# Autodesk Inventor assembly: main_assembly
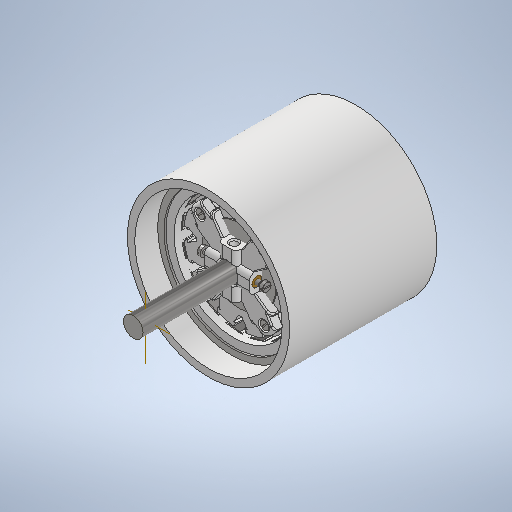
[picture p0: Inventor's stored thumbnail of the model, 512x512]
Saved by Autodesk Inventor 2025 (Build 290162000, 162)
## iProperties
Created: 2026-08-03
Part Number: main_assembly
Document SubType Name: Assembly
Designer: zzapa
Author: zzapa
## Documents named in this file (13)
- C:\Users\zzapa\Desktop\Projekty\elektronika\engine-project\model\assemblies\main_assembly.iam
- C:\Users\zzapa\Desktop\Projekty\elektronika\engine-project\model\parts\stator_metal.ipt
- C:\Users\zzapa\Desktop\Projekty\elektronika\engine-project\model\assemblies\magnet_ring_assembly.iam
- C:\Users\zzapa\Desktop\Projekty\elektronika\engine-project\model\parts\casing_cylindrical.ipt
- C:\Users\zzapa\Desktop\Projekty\elektronika\engine-project\model\parts\rotor_plastic.ipt
- C:\Users\zzapa\Desktop\Projekty\elektronika\engine-project\model\assemblies\rotor_core.iam
- C:\Users\zzapa\Desktop\Projekty\elektronika\engine-project\model\parts\shaft.ipt
- C:\Users\zzapa\Documents\Inventor\Content Center Files\R2025\pl-PL\GB 809-88 A\Nut GB 809 A M2,5 x 6.ipt
- C:\Users\zzapa\Documents\Inventor\Content Center Files\R2025\pl-PL\CNS 4355\CNS 4355 - M 2 x 6.ipt
- C:\Users\zzapa\Desktop\Projekty\elektronika\engine-project\model\parts\shaft_lock_1.ipt
- C:\Users\zzapa\Documents\Inventor\Content Center Files\R2025\pl-PL\GB 809-88 A\Nut GB 809 A M2 x 3.ipt
- C:\Users\zzapa\Documents\Inventor\Content Center Files\R2025\pl-PL\CNS 4355\CNS 4355 - M 2 x 8.ipt
- C:\Users\zzapa\Desktop\Projekty\elektronika\engine-project\model\parts\shaft_lock_2.ipt
## Components (32 placed, 12 different names)
1. stator_metal:1 — Zestawiające:1, Kątowe:1
2. magnet_ring_assembly:1 [sub-assembly] — Zestawiające:2
3. casing_cylindrical:1 — Zestawiające:3, Kątowe:2
4. rotor_plastic:1 — Zestawiające:4, Zestawiające:7, Zestawiające:8, Zestawiające:9, Zestawiające:10, Równoległe:1, Równoległe:2, Równoległe:3, Równoległe:4, Zestawiające:31, Zestawiające:40, Zestawiające:41, Zestawiające:42, Zestawiające:43, Zestawiające:44, Równoległe:5, Równoległe:6, Równoległe:7, Równoległe:8, Kątowe:13, Zestawiające:52
5. rotor_core:1 [sub-assembly] — Zestawiające:5, Zestawiające:30
6. shaft:1 — Zestawiające:6, Zestawiające:28, Styczny:1, Styczny:2, Zestawiające:50
7. Nut GB/T 809-1988 Type A M2,5x6:1 — Kątowe:3, Zestawiające:7, Równoległe:3
8. Nut GB/T 809-1988 Type A M2,5x6:2 — Kątowe:4, Zestawiające:9, Równoległe:1
9. Nut GB/T 809-1988 Type A M2,5x6:3 — Kątowe:5, Zestawiające:8, Równoległe:2, Zestawiające:51
10. Nut GB/T 809-1988 Type A M2,5x6:4 — Kątowe:6, Zestawiające:10, Równoległe:4
11. shaft_lock_1:1 — Zestawiające:28, Zestawiające:30, Zestawiające:31, Zestawiające:32, Zestawiające:33, Zestawiające:34, Zestawiające:35, Zestawiające:36, Zestawiające:37, Zestawiające:38, Zestawiające:39, Zestawiające:40, Zestawiające:45, Zestawiające:46, Równoległe:9, Równoległe:10
12. CNS 4355 M 2 x 6:5 — Zestawiające:32, Zestawiające:36
13. CNS 4355 M 2 x 6:6 — Zestawiające:35, Zestawiające:39
14. CNS 4355 M 2 x 6:7 — Zestawiające:34, Zestawiające:38
15. CNS 4355 M 2 x 6:8 — Zestawiające:33, Zestawiające:37
16. Nut GB/T 809-1988 Type A M2,5x6:6 — Zestawiające:42, Równoległe:7
17. Nut GB/T 809-1988 Type A M2,5x6:7 — Zestawiające:44, Równoległe:6
18. Nut GB/T 809-1988 Type A M2,5x6:8 — Zestawiające:43, Równoległe:5
19. Nut GB/T 809-1988 Type A M2,5x6:9 — Zestawiające:41, Równoległe:8
20. Nut GB/T 809-1988 Type A M2x3:1 — Zestawiające:45, Równoległe:10, Zestawiające:47
21. Nut GB/T 809-1988 Type A M2x3:2 — Zestawiające:46, Równoległe:9, Zestawiające:48
22. CNS 4355 M 2 x 8:1 — Zestawiające:48, Równoległe:11
23. CNS 4355 M 2 x 8:2 — Zestawiające:47, Zestawiające:49
24. shaft_lock_2:1 — Zestawiające:50, Zestawiające:51, Zestawiające:52, Zestawiające:53, Zestawiające:54, Równoległe:12, Równoległe:13, Zestawiające:58, Zestawiające:59, Zestawiające:60, Zestawiające:61, Zestawiające:62, Zestawiające:63, Zestawiające:64, Zestawiające:65
25. Nut GB/T 809-1988 Type A M2x3:3 — Zestawiające:53, Równoległe:13, Zestawiające:57
26. Nut GB/T 809-1988 Type A M2x3:4 — Zestawiające:54, Równoległe:12, Zestawiające:56
27. CNS 4355 M 2 x 8:3 — Zestawiające:55, Zestawiające:57
28. CNS 4355 M 2 x 8:4 — Równoległe:14, Zestawiające:56
29. CNS 4355 M 2 x 6:9 — Zestawiające:60, Zestawiające:63
30. CNS 4355 M 2 x 6:10 — Zestawiające:61, Zestawiające:64
31. CNS 4355 M 2 x 6:11 — Zestawiające:59, Zestawiające:65
32. CNS 4355 M 2 x 6:12 — Zestawiające:58, Zestawiające:62
## Relationships (72: Mate 47, Flush 14, Angle 9, Tangent 2)
- Zestawiające:1 [Mate]: stator_metal:1
- Kątowe:1 [Angle] (0 deg): stator_metal:1
- Zestawiające:2 [Mate]: magnet_ring_assembly:1
- Zestawiające:3 [Mate]: casing_cylindrical:1
- Kątowe:2 [Angle] (0 deg): casing_cylindrical:1
- Zestawiające:4 [Mate]: rotor_plastic:1
- Zestawiające:5 [Mate]: rotor_core:1
- Zestawiające:6 [Mate]: shaft:1
- Kątowe:3 [Angle] (0 deg): Nut GB/T 809-1988 Type A M2,5x6:1
- Kątowe:4 [Angle] (0 deg): Nut GB/T 809-1988 Type A M2,5x6:2
- Kątowe:5 [Angle] (0 deg): Nut GB/T 809-1988 Type A M2,5x6:3
- Kątowe:6 [Angle] (0 deg): Nut GB/T 809-1988 Type A M2,5x6:4
- Zestawiające:7 [Mate]: rotor_plastic:1 ↔ Nut GB/T 809-1988 Type A M2,5x6:1
- Zestawiające:8 [Mate]: rotor_plastic:1 ↔ Nut GB/T 809-1988 Type A M2,5x6:3
- Zestawiające:9 [Mate]: rotor_plastic:1 ↔ Nut GB/T 809-1988 Type A M2,5x6:2
- Zestawiające:10 [Mate]: rotor_plastic:1 ↔ Nut GB/T 809-1988 Type A M2,5x6:4
- Równoległe:1 [Flush]: rotor_plastic:1 ↔ Nut GB/T 809-1988 Type A M2,5x6:2
- Równoległe:2 [Flush]: rotor_plastic:1 ↔ Nut GB/T 809-1988 Type A M2,5x6:3
- Równoległe:3 [Flush]: rotor_plastic:1 ↔ Nut GB/T 809-1988 Type A M2,5x6:1
- Równoległe:4 [Flush]: rotor_plastic:1 ↔ Nut GB/T 809-1988 Type A M2,5x6:4
- Zestawiające:28 [Mate]: shaft:1 ↔ shaft_lock_1:1
- Zestawiające:30 [Mate]: rotor_core:1 ↔ shaft_lock_1:1
- Zestawiające:31 [Mate]: rotor_plastic:1 ↔ shaft_lock_1:1
- Zestawiające:32 [Mate]: shaft_lock_1:1 ↔ CNS 4355 M 2 x 6:5
- Zestawiające:33 [Mate]: shaft_lock_1:1 ↔ CNS 4355 M 2 x 6:8
- Zestawiające:34 [Mate]: shaft_lock_1:1 ↔ CNS 4355 M 2 x 6:7
- Zestawiające:35 [Mate]: shaft_lock_1:1 ↔ CNS 4355 M 2 x 6:6
- Zestawiające:36 [Mate]: shaft_lock_1:1 ↔ CNS 4355 M 2 x 6:5
- Zestawiające:37 [Mate]: shaft_lock_1:1 ↔ CNS 4355 M 2 x 6:8
- Zestawiające:38 [Mate]: shaft_lock_1:1 ↔ CNS 4355 M 2 x 6:7
- Zestawiające:39 [Mate]: shaft_lock_1:1 ↔ CNS 4355 M 2 x 6:6
- Zestawiające:40 [Mate]: rotor_plastic:1 ↔ shaft_lock_1:1
- Zestawiające:41 [Mate]: rotor_plastic:1 ↔ Nut GB/T 809-1988 Type A M2,5x6:9
- Zestawiające:42 [Mate]: rotor_plastic:1 ↔ Nut GB/T 809-1988 Type A M2,5x6:6
- Zestawiające:43 [Mate]: rotor_plastic:1 ↔ Nut GB/T 809-1988 Type A M2,5x6:8
- Zestawiające:44 [Mate]: rotor_plastic:1 ↔ Nut GB/T 809-1988 Type A M2,5x6:7
- Równoległe:5 [Flush]: rotor_plastic:1 ↔ Nut GB/T 809-1988 Type A M2,5x6:8
- Równoległe:6 [Flush]: rotor_plastic:1 ↔ Nut GB/T 809-1988 Type A M2,5x6:7
- Równoległe:7 [Flush]: rotor_plastic:1 ↔ Nut GB/T 809-1988 Type A M2,5x6:6
- Równoległe:8 [Flush]: rotor_plastic:1 ↔ Nut GB/T 809-1988 Type A M2,5x6:9
- Kątowe:13 [Angle] (0 deg): rotor_plastic:1
- Zestawiające:45 [Mate]: shaft_lock_1:1 ↔ Nut GB/T 809-1988 Type A M2x3:1
- Zestawiające:46 [Mate]: shaft_lock_1:1 ↔ Nut GB/T 809-1988 Type A M2x3:2
- Równoległe:9 [Flush]: shaft_lock_1:1 ↔ Nut GB/T 809-1988 Type A M2x3:2
- Równoległe:10 [Flush]: shaft_lock_1:1 ↔ Nut GB/T 809-1988 Type A M2x3:1
- Zestawiające:47 [Mate]: Nut GB/T 809-1988 Type A M2x3:1 ↔ CNS 4355 M 2 x 8:2
- Zestawiające:48 [Mate]: Nut GB/T 809-1988 Type A M2x3:2 ↔ CNS 4355 M 2 x 8:1
- Kątowe:14 [Angle] (0 deg)
- Styczny:1 [Tangent]: shaft:1
- Kątowe:15 [Angle] (0 deg)
- Styczny:2 [Tangent]: shaft:1
- Zestawiające:49 [Mate]: CNS 4355 M 2 x 8:2
- Równoległe:11 [Flush]: CNS 4355 M 2 x 8:1
- Zestawiające:50 [Mate]: shaft:1 ↔ shaft_lock_2:1
- Zestawiające:51 [Mate]: Nut GB/T 809-1988 Type A M2,5x6:3 ↔ shaft_lock_2:1
- Zestawiające:52 [Mate]: rotor_plastic:1 ↔ shaft_lock_2:1
- Zestawiające:53 [Mate]: shaft_lock_2:1 ↔ Nut GB/T 809-1988 Type A M2x3:3
- Zestawiające:54 [Mate]: shaft_lock_2:1 ↔ Nut GB/T 809-1988 Type A M2x3:4
- Równoległe:12 [Flush]: shaft_lock_2:1 ↔ Nut GB/T 809-1988 Type A M2x3:4
- Równoległe:13 [Flush]: shaft_lock_2:1 ↔ Nut GB/T 809-1988 Type A M2x3:3
- Równoległe:14 [Flush]: CNS 4355 M 2 x 8:4
- Zestawiające:55 [Mate]: CNS 4355 M 2 x 8:3
- Zestawiające:56 [Mate]: Nut GB/T 809-1988 Type A M2x3:4 ↔ CNS 4355 M 2 x 8:4
- Zestawiające:57 [Mate]: Nut GB/T 809-1988 Type A M2x3:3 ↔ CNS 4355 M 2 x 8:3
- Zestawiające:58 [Mate]: shaft_lock_2:1 ↔ CNS 4355 M 2 x 6:12
- Zestawiające:59 [Mate]: shaft_lock_2:1 ↔ CNS 4355 M 2 x 6:11
- Zestawiające:60 [Mate]: shaft_lock_2:1 ↔ CNS 4355 M 2 x 6:9
- Zestawiające:61 [Mate]: shaft_lock_2:1 ↔ CNS 4355 M 2 x 6:10
- Zestawiające:62 [Mate]: shaft_lock_2:1 ↔ CNS 4355 M 2 x 6:12
- Zestawiające:63 [Mate]: shaft_lock_2:1 ↔ CNS 4355 M 2 x 6:9
- Zestawiające:64 [Mate]: shaft_lock_2:1 ↔ CNS 4355 M 2 x 6:10
- Zestawiające:65 [Mate]: shaft_lock_2:1 ↔ CNS 4355 M 2 x 6:11
